# Autodesk Inventor assembly: liftidea1
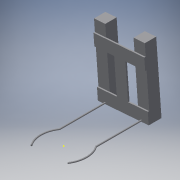
[picture p0: Inventor's stored thumbnail of the model, 180x180]
Saved by Autodesk Inventor 2017 (Build 210142000, 142)
## iProperties
Created: 2017-05-30
Part Number: liftidea1
Document SubType Name: Assembly
Designer: User
Author: User
## Documents named in this file (4)
- C:\Robotics\CAD\2016-17_CAD\liftidea1.iam
- C:\Robotics\CAD\2016-17_CAD\backplatelift.ipt
- C:\Robotics\CAD\2016-17_CAD\outlineslides.ipt
- C:\Robotics\CAD\2016-17_CAD\LiftBallHolder.ipt
## Components (4 placed, 3 different names)
1. backplatelift:1 — Mate:11, Flush:17, Flush:18, Mate:12, Flush:19, Flush:20, Mate:13, Mate:14, Mate:15, Flush:21, Flush:22
2. outlineslides:1 — Mate:11, Flush:17, Flush:18, Flush:21
3. outlineslides:2 — Mate:12, Flush:19, Flush:20, Flush:22
4. LiftBallHolder:1 — Mate:13, Mate:14, Mate:15
## Relationships (11: Flush 6, Mate 5)
- Mate:11: backplatelift:1 ↔ outlineslides:1
- Flush:17: backplatelift:1 ↔ outlineslides:1
- Flush:18: backplatelift:1 ↔ outlineslides:1
- Mate:12: backplatelift:1 ↔ outlineslides:2
- Flush:19: backplatelift:1 ↔ outlineslides:2
- Flush:20: backplatelift:1 ↔ outlineslides:2
- Mate:13: backplatelift:1 ↔ LiftBallHolder:1
- Mate:14: backplatelift:1 ↔ LiftBallHolder:1
- Mate:15: backplatelift:1 ↔ LiftBallHolder:1
- Flush:21: backplatelift:1 ↔ outlineslides:1
- Flush:22: backplatelift:1 ↔ outlineslides:2
